# Autodesk Inventor assembly: Assembly1
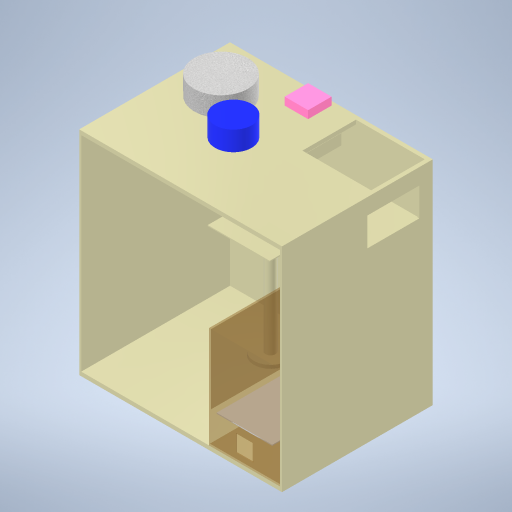
[picture p0: Inventor's stored thumbnail of the model, 512x512]
Saved by Autodesk Inventor 2023 (Build 270158000, 158)
## iProperties
Created: 2022-05-16
Part Number: Assembly1
Document SubType Name: Assembly
Designer: techv
Author: techv
## Documents named in this file (7)
- D:\Projects\P_Baker Bot\Design\Assembly1.iam
- D:\Projects\P_Baker Bot\Design\Outer Casing.ipt
- D:\Projects\P_Baker Bot\Design\Flour Container.ipt
- D:\Projects\P_Baker Bot\Design\water container.ipt
- D:\Projects\P_Baker Bot\Design\oil container.ipt
- D:\Projects\P_Baker Bot\Juicer\mesh body.ipt
- D:\Projects\P_Baker Bot\Design\STL\hot box.iam
## Components (6 placed, 6 different names)
1. Outer Casing:1 — Mate:1, Mate:2, Mate:3, Mate:4, Mate:5, Mate:6, Mate:7, Mate:8, Flush:1, Mate:9
2. Flour Container:1 — Mate:1, Mate:2
3. water container:1 — Mate:3, Mate:4
4. oil container:1 — Mate:5, Mate:6, Mate:7
5. mesh body:1
6. hot box:1 [sub-assembly] — Mate:8, Flush:1, Mate:9
## Relationships (10: Mate 9, Flush 1)
- Mate:1: Outer Casing:1 ↔ Flour Container:1
- Mate:2: Outer Casing:1 ↔ Flour Container:1
- Mate:3: Outer Casing:1 ↔ water container:1
- Mate:4: Outer Casing:1 ↔ water container:1
- Mate:5: Outer Casing:1 ↔ oil container:1
- Mate:6: Outer Casing:1 ↔ oil container:1
- Mate:7: Outer Casing:1 ↔ oil container:1
- Mate:8: Outer Casing:1 ↔ hot box:1
- Flush:1: Outer Casing:1 ↔ hot box:1
- Mate:9: Outer Casing:1 ↔ hot box:1
